# Autodesk Inventor assembly: Pin-Assembly
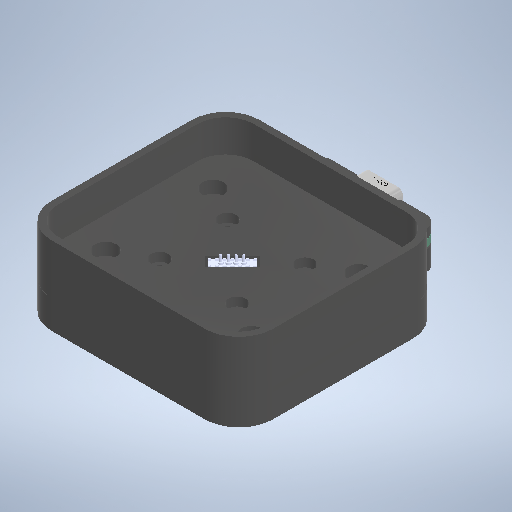
[picture p0: Inventor's stored thumbnail of the model, 512x512]
Saved by Autodesk Inventor 2025 (Build 290162000, 162)
## iProperties
Created: 2025-03-04
Part Number: Pin-Assembly
Document SubType Name: Assembly
Designer: maxsm
Author: maxsm
## iProperties of the stored document R_0402_1005Metric.iam
Created: 2025-04-26
Part Number: R_0402_1005Metric
Document SubType Name: Assembly
Designer: maxsm
Author: maxsm
## iProperties of the stored document R_0402_1005Metric.ipt
Created: 2025-04-26
Part Number: R_0402_1005Metric
Material: Generic
Document SubType Name: Modeling
Designer: maxsm
Density: 1 g/cm^3
Appearance: Default
Author: maxsm
## iProperties of the stored document Interposer-PCB.iam
Company: Kicad
Created: 2025-04-26
Part Number: pin-interposer 1
Description: KiCad electronic assembly
Document SubType Name: Assembly
Designer: maxsm
Authority: Unknown
Sending System: KiCad to STEP converter
Preprocessor: Open CASCADE STEP processor 7.7
Title: pin-interposer.step
Author: Pcbnew
## iProperties of the stored document 854-22-004-10-001101.ipt
Created: 2025-03-04
Part Number: 854-22-004-10-001101
Material: Generic
Document SubType Name: Modeling
Designer: maxsm
Density: 1 g/cm^3
Appearance: Default
Author: maxsm
## iProperties of the stored document USB-SMD_GT-USB-7010AN.ipt
Created: 2025-04-26
Part Number: USB-SMD_GT-USB-7010AN
Material: Generic
Document SubType Name: Modeling
Designer: maxsm
Density: 1 g/cm^3
Appearance: Default
Author: maxsm
## iProperties of the stored document USB-SMD_GT-USB-7010AN.iam
Created: 2025-04-26
Part Number: USB-SMD_GT-USB-7010AN
Document SubType Name: Assembly
Designer: maxsm
Author: maxsm
## iProperties of the stored document _autosave-pin-interposer PCB.ipt
Created: 2025-04-26
Part Number: _autosave-pin-interposer PCB
Material: Generic
Document SubType Name: Modeling
Designer: maxsm
Density: 1 g/cm^3
Appearance: Default
Author: maxsm
## iProperties of the stored document 854-22-004-10-001101.iam
Created: 2025-03-04
Part Number: 854-22-004-10-001101
Document SubType Name: Assembly
Designer: maxsm
Author: maxsm
## Documents named in this file (13)
- C:\Users\maxsm\root\OpenPin\interposer\prints\v2\Pin-Assembly.iam
- C:\Users\maxsm\root\OpenPin\interposer\prints\v2\Pin-Low-Fidelity.ipt
- **C:\Users\maxsm\root\OpenPin\interposer\prints\v2\Pin-Assembly.iam*LocalDocs*xAaaaa4baAaaaaaaaAaaaad2mSc*Interposer-PCB.iam
- C:\Users\maxsm\root\OpenPin\interposer\prints\v2\Pin-Cradle.ipt
- C:\Users\maxsm\root\OpenPin\interposer\prints\v2\Pin-Base.ipt
- **C:\Users\maxsm\root\OpenPin\interposer\prints\v2\Pin-Assembly.iam*LocalDocs*xAaaaaxdaAaaaaaaaAaaaqddbFf*R_0402_1005Metric.iam
- **C:\Users\maxsm\root\OpenPin\interposer\prints\v2\Pin-Assembly.iam*LocalDocs*xAaaaa4daAaaaaaaaAaaaqigvFc*R_0402_1005Metric.ipt
- **C:\Users\maxsm\root\OpenPin\interposer\prints\v2\Pin-Assembly.iam*LocalDocs*xAaaaqscaAaaaaaaaAaaaalt4De*854-22-004-10-001101.iam
- **C:\Users\maxsm\root\OpenPin\interposer\prints\v2\Pin-Assembly.iam*LocalDocs*xAaaaq1aaAaaaaaaaAaaaavdm1h*USB-SMD_GT-USB-7010AN.iam
- **C:\Users\maxsm\root\OpenPin\interposer\prints\v2\Pin-Assembly.iam*LocalDocs*xAaaaqlcaAaaaaaaaAaaaqgnfBe*_autosave-pin-interposer PCB.ipt
- **C:\Users\maxsm\root\OpenPin\interposer\prints\v2\Pin-Assembly.iam*LocalDocs*xAaaaancaAaaaaaaaAaaaqxtpDh*854-22-004-10-001101.ipt
- **C:\Users\maxsm\root\OpenPin\interposer\prints\v2\Pin-Assembly.iam*LocalDocs*xAaaaq5baAaaaaaaaAaaaa1gh1f*USB-SMD_GT-USB-7010AN.ipt
- C:\Users\maxsm\root\OpenPin\interposer\prints\v2\Interposer-PCB.step
## Components (4 placed, 4 different names)
1. Pin-Low-Fidelity:1 — Mate:1, Mate:2, Mate:3
2. Interposer-PCB:1 [sub-assembly] — Mate:4, Mate:5, Flush:1
3. Pin-Cradle:1 — Mate:1, Mate:2, Mate:3, Mate:4, Mate:5, Flush:1, Mate:6, Mate:7, Mate:8
4. Pin-Base:1 — Mate:6, Mate:7, Mate:8
## Relationships (9: Mate 8, Flush 1)
- Mate:1 (0.5 mm): Pin-Low-Fidelity:1 ↔ Pin-Cradle:1
- Mate:2: Pin-Low-Fidelity:1 ↔ Pin-Cradle:1
- Mate:3 (0.5 mm): Pin-Low-Fidelity:1 ↔ Pin-Cradle:1
- Mate:4: Interposer-PCB:1 ↔ Pin-Cradle:1
- Mate:5: Interposer-PCB:1 ↔ Pin-Cradle:1
- Flush:1: Interposer-PCB:1 ↔ Pin-Cradle:1
- Mate:6: Pin-Cradle:1 ↔ Pin-Base:1
- Mate:7: Pin-Cradle:1 ↔ Pin-Base:1
- Mate:8: Pin-Cradle:1 ↔ Pin-Base:1
